# Autodesk Inventor assembly: Assembly_LampeSolaire2
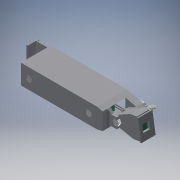
[picture p0: Inventor's stored thumbnail of the model, 180x180]
Saved by Autodesk Inventor 2019 (Build 230136000, 136)
## iProperties
Created: 2020-09-16
Part Number: Assembly_LampeSolaire2
Document SubType Name: Assembly
Designer: nicolas
Author: nicolas
## Documents named in this file (22)
- C:\Workspace\3D\Cad\LampeSolaire2\Assembly_LampeSolaire2.iam
- C:\Workspace\3D\Cad\LampeSolaire2\LampeSolaire2.iam
- C:\Workspace\3D\Cad\LampeSolaire2\ChargerModule.iam
- C:\Workspace\3D\Cad\LampeSolaire2\ledsAdapter_base.ipt
- C:\Workspace\3D\Cad\LampeSolaire2\LampeSolaire2_Casing.ipt
- C:\Workspace\3D\Cad\LampeSolaire2\LampeSolaire2_LedAmoviblePart.ipt
- C:\Workspace\3D\Cad\Screws\Hex_m5\M5x0.8xL.ipt
- C:\Workspace\3D\Cad\Screws\Hex_m5\M5x0.8xL\M5x0.8x35.ipt
- C:\Workspace\3D\Cad\Screws\wing_nuts\WNM5.ipt
- C:\Workspace\3D\Cad\Screws\hexagonal-bolts\ledAdapter.ipt
- C:\Workspace\3D\Cad\Screws\Hex_m5\M5x0.8xL_Partial_L2.ipt
- C:\Workspace\3D\Cad\LampeSolaire2\LampeSolaire2_LedAmoviblePart_Cover.ipt
- C:\Workspace\3D\Cad\Screws\Hex_m3\M3x0.8xL.ipt
- C:\Workspace\3D\Cad\Nuts\Nut_Generic\Ec 6p ISO 4032-M3.ipt
- C:\Workspace\3D\Cad\Nuts\Nut_Generic.ipt
- C:\Workspace\3D\Cad\Nuts\Nut_Generic\Ec 6p ISO 4032-M5.ipt
- C:\Workspace\3D\Cad\LampeSolaire2\LampeSolaire2_Casing_Cover.ipt
- C:\Workspace\3D\Cad\LampeSolaire2\Rope.ipt
- C:\Workspace\3D\Cad\Screws\Hex_m3\M3x0.8xL\M3x0.8x20.ipt
- C:\Workspace\3D\Cad\Washers\SpringWasher\Spring Washer M5.ipt
- C:\Workspace\3D\Cad\Washers\SpringWasher.ipt
- C:\Workspace\3D\Cad\Screws\Hex_m5\M5x0.8xL_Partial_L2\M5x0.8x40_Partial_16.ipt
## Components (21 placed, 16 different names)
1. LampeSolaire2_Casing:1 — Mate:2, Mate:27, Mate:29, Mate:30, Mate:31, Mate:32, Mate:45, Mate:46, Mate:47, Mate:51, Mate:64, Mate:65, Slider:1, Mate:66, Mate:68, Mate:70, Mate:71
2. LampeSolaire2_Casing_Cover:1 — Slider:1
3. LampeSolaire2_LedAmoviblePart:1 — Mate:2, Cylindrical:1, Mate:52, Cylindrical:4, Flush:2, Mate:54, Mate:56, Mate:57, Mate:60, Mate:69
4. LampeSolaire2_LedAmoviblePart_Cover:1 — Flush:2, Mate:54, Mate:59, Mate:61
5. LampeSolaire2:1 [sub-assembly] — Mate:37, Mate:38, Mate:40, Mate:41, Mate:44
6. ChargerModule:1 [sub-assembly] — Mate:42, Mate:43, Mate:44, Mate:45
7. ledAdapter:3
8. ledsAdapter_base:1 — Mate:52, Cylindrical:4, Mate:73
9. Ec 6p ISO 4032-M5:2 — Mate:33, Mate:40
10. Ec 6p ISO 4032-M5:3 — Mate:39, Mate:41
11. Ec 6p ISO 4032-M5:4 — Mate:36, Mate:47
12. Ec 6p ISO 4032-M5:5 — Mate:35, Mate:46
13. Ec 6p ISO 4032-M3:1 — Mate:59, Mate:62
14. Ec 6p ISO 4032-M3:6 — Mate:72, Mate:73
15. M5x0.8x40_Partial_16:1 — Mate:27, Cylindrical:1, Mate:50, Mate:67, Mate:69, Mate:70
16. M5x0.8x35:2 — Mate:29, Mate:30, Mate:33, Mate:35, Mate:37, Mate:42
17. M5x0.8x35:3 — Mate:31, Mate:32, Mate:36, Mate:38, Mate:39, Mate:43
18. M3x0.8x20:1 — Mate:56, Mate:57, Mate:60, Mate:61, Mate:62, Mate:72
19. WNM5:1 — Mate:50, Mate:51
20. Spring Washer M5:1 — Mate:67, Mate:68
21. Rope:1 — Mate:66, Mate:71
## Relationships (45: Mate 40, CylindricalJoint 2, WeldJoint 1, Flush 1, TranslationJoint 1)
- Mate:2: LampeSolaire2_Casing:1 ↔ LampeSolaire2_LedAmoviblePart:1
- Mate:27: LampeSolaire2_Casing:1 ↔ M5x0.8x40_Partial_16:1
- Mate:29: LampeSolaire2_Casing:1 ↔ M5x0.8x35:2
- Mate:30: LampeSolaire2_Casing:1 ↔ M5x0.8x35:2
- Mate:31: LampeSolaire2_Casing:1 ↔ M5x0.8x35:3
- Mate:32: LampeSolaire2_Casing:1 ↔ M5x0.8x35:3
- Mate:33: Ec 6p ISO 4032-M5:2 ↔ M5x0.8x35:2
- Mate:35: Ec 6p ISO 4032-M5:5 ↔ M5x0.8x35:2
- Mate:36: Ec 6p ISO 4032-M5:4 ↔ M5x0.8x35:3
- Mate:37: LampeSolaire2:1 ↔ M5x0.8x35:2
- Mate:38: LampeSolaire2:1 ↔ M5x0.8x35:3
- Mate:39: Ec 6p ISO 4032-M5:3 ↔ M5x0.8x35:3
- Mate:40: LampeSolaire2:1 ↔ Ec 6p ISO 4032-M5:2
- Mate:41: LampeSolaire2:1 ↔ Ec 6p ISO 4032-M5:3
- Mate:42: ChargerModule:1 ↔ M5x0.8x35:2
- Mate:43: ChargerModule:1 ↔ M5x0.8x35:3
- Mate:44: LampeSolaire2:1 ↔ ChargerModule:1
- Mate:45 (10 mm): LampeSolaire2_Casing:1 ↔ ChargerModule:1
- Cylindrical:1: LampeSolaire2_LedAmoviblePart:1 ↔ M5x0.8x40_Partial_16:1
- [WeldJoint]: LampeSolaire2_LedAmoviblePart:1 ↔ ledAdapter:3
- Mate:46: LampeSolaire2_Casing:1 ↔ Ec 6p ISO 4032-M5:5
- Mate:47: LampeSolaire2_Casing:1 ↔ Ec 6p ISO 4032-M5:4
- Mate:50: M5x0.8x40_Partial_16:1 ↔ WNM5:1
- Mate:51: LampeSolaire2_Casing:1 ↔ WNM5:1
- Mate:52: LampeSolaire2_LedAmoviblePart:1 ↔ ledsAdapter_base:1
- Cylindrical:4: LampeSolaire2_LedAmoviblePart:1 ↔ ledsAdapter_base:1
- Flush:2: LampeSolaire2_LedAmoviblePart:1 ↔ LampeSolaire2_LedAmoviblePart_Cover:1
- Mate:54: LampeSolaire2_LedAmoviblePart:1 ↔ LampeSolaire2_LedAmoviblePart_Cover:1
- Mate:56: LampeSolaire2_LedAmoviblePart:1 ↔ M3x0.8x20:1
- Mate:57: LampeSolaire2_LedAmoviblePart:1 ↔ M3x0.8x20:1
- Mate:59: LampeSolaire2_LedAmoviblePart_Cover:1 ↔ Ec 6p ISO 4032-M3:1
- Mate:60: LampeSolaire2_LedAmoviblePart:1 ↔ M3x0.8x20:1
- Mate:61: LampeSolaire2_LedAmoviblePart_Cover:1 ↔ M3x0.8x20:1
- Mate:62: Ec 6p ISO 4032-M3:1 ↔ M3x0.8x20:1
- Mate:64: LampeSolaire2_Casing:1
- Mate:65: LampeSolaire2_Casing:1
- Slider:1 [TranslationJoint]: LampeSolaire2_Casing:1 ↔ LampeSolaire2_Casing_Cover:1
- Mate:66: LampeSolaire2_Casing:1 ↔ Rope:1
- Mate:67: M5x0.8x40_Partial_16:1 ↔ Spring Washer M5:1
- Mate:68: LampeSolaire2_Casing:1 ↔ Spring Washer M5:1
- Mate:69: LampeSolaire2_LedAmoviblePart:1 ↔ M5x0.8x40_Partial_16:1
- Mate:70: LampeSolaire2_Casing:1 ↔ M5x0.8x40_Partial_16:1
- Mate:71: LampeSolaire2_Casing:1 ↔ Rope:1
- Mate:72: Ec 6p ISO 4032-M3:6 ↔ M3x0.8x20:1
- Mate:73: ledsAdapter_base:1 ↔ Ec 6p ISO 4032-M3:6
